# Autodesk Inventor assembly: Hauptmodul
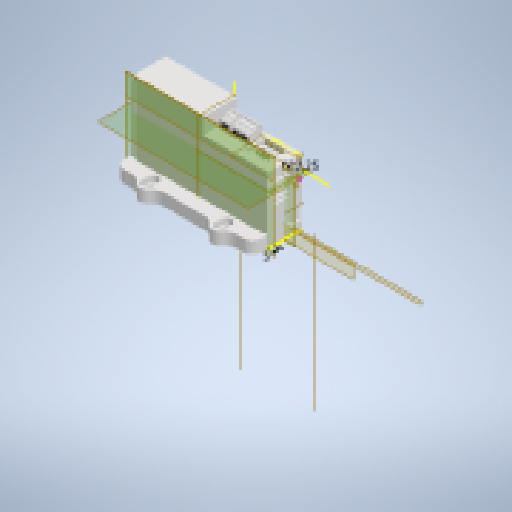
[picture p0: Inventor's stored thumbnail of the model, 512x512]
Saved by Autodesk Inventor 2025.2 (Build 292293000, 293)
## iProperties
Created: 2025-11-03
Part Number: Hauptmodul
Document SubType Name: Assembly
Designer: leowa
Author: leowa
## Documents named in this file (6)
- C:\Users\leowa\OneDrive - Fachhochschule Aachen\FH\8. Semester\CANTram-Framework\Inventor CAD\Workspaces\Arbeitsbereich\Module\Hauptmodul.iam
- C:\Users\leowa\OneDrive - Fachhochschule Aachen\FH\8. Semester\CANTram-Framework\Inventor CAD\Workspaces\Arbeitsbereich\Platinen\Hauptmodul\Hauptmodul\Hauptmodul.iam
- C:\Users\leowa\OneDrive - Fachhochschule Aachen\FH\8. Semester\CANTram-Framework\Inventor CAD\Workspaces\Arbeitsbereich\Kaufteile\Terminalstecker 2fach\0395000002.iam
- C:\Users\leowa\OneDrive - Fachhochschule Aachen\FH\8. Semester\CANTram-Framework\Inventor CAD\Workspaces\Arbeitsbereich\Kaufteile\Terminalstecker 4fach\0395000004.iam
- C:\Users\leowa\OneDrive - Fachhochschule Aachen\FH\8. Semester\CANTram-Framework\Inventor CAD\Workspaces\Arbeitsbereich\Gehäuse\Hauptmodul Gehäuse V2.ipt
- C:\Users\leowa\OneDrive - Fachhochschule Aachen\FH\8. Semester\CANTram-Framework\Inventor CAD\Workspaces\Arbeitsbereich\Gehäuse\Hauptmodul Deckel V2.ipt
## Components (5 placed, 5 different names)
1. Hauptmodul:1 [sub-assembly] — Passend:6, Passend:7, Passend:8, Passend:9, Passend:10, Passend:11, Passend:12, Passend:13, Passend:14
2. 0395000002:1 [sub-assembly] — Passend:7, Passend:9, Passend:11
3. 0395000004:1 [sub-assembly] — Passend:6, Passend:8, Passend:10
4. Hauptmodul Gehäuse V2:1 — Passend:12, Passend:13, Passend:14, Fluchtend:3, Fluchtend:4, Passend:15
5. Hauptmodul Deckel V2:1 — Fluchtend:3, Fluchtend:4, Passend:15
## Relationships (12: Mate 10, Flush 2)
- Passend:6 [Mate]: Hauptmodul:1 ↔ 0395000004:1
- Passend:7 [Mate]: Hauptmodul:1 ↔ 0395000002:1
- Passend:8 [Mate]: Hauptmodul:1 ↔ 0395000004:1
- Passend:9 [Mate]: Hauptmodul:1 ↔ 0395000002:1
- Passend:10 [Mate]: Hauptmodul:1 ↔ 0395000004:1
- Passend:11 [Mate]: Hauptmodul:1 ↔ 0395000002:1
- Passend:12 [Mate]: Hauptmodul:1 ↔ Hauptmodul Gehäuse V2:1
- Passend:13 [Mate]: Hauptmodul:1 ↔ Hauptmodul Gehäuse V2:1
- Passend:14 [Mate] (1 mm): Hauptmodul:1 ↔ Hauptmodul Gehäuse V2:1
- Fluchtend:3 [Flush]: Hauptmodul Gehäuse V2:1 ↔ Hauptmodul Deckel V2:1
- Fluchtend:4 [Flush]: Hauptmodul Gehäuse V2:1 ↔ Hauptmodul Deckel V2:1
- Passend:15 [Mate]: Hauptmodul Gehäuse V2:1 ↔ Hauptmodul Deckel V2:1
